# Autodesk Inventor assembly: BATTERY ASSEMBLY
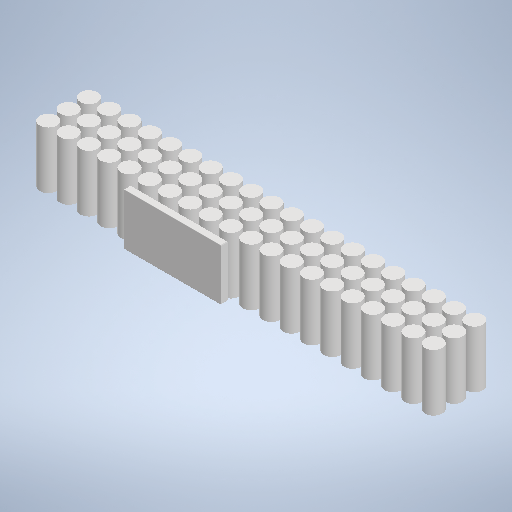
[picture p0: Inventor's stored thumbnail of the model, 512x512]
Saved by Autodesk Inventor 2025.2 (Build 292293000, 293)
## iProperties
Created: 2025-03-22
Part Number: BATTERY ASSEMBLY
Document SubType Name: Assembly
Designer: Mathias
Author: Mathias
## Documents named in this file (3)
- C:\Users\Mathias\Desktop\Projekt Olkassa\Autodesk-inventor-filesharing\BATTERY ASSEMBLY.iam
- C:\Users\Mathias\Desktop\Projekt Olkassa\Autodesk-inventor-filesharing\21700.ipt
- C:\Users\Mathias\Desktop\Projekt Olkassa\Autodesk-inventor-filesharing\BMS.ipt
## Components (61 placed, 2 different names)
1. BMS:1
2. 21700:1
3. 21700:2
4. 21700:3
5. 21700:4
6. 21700:5
7. 21700:6
8. 21700:7
9. 21700:8
10. 21700:9
11. 21700:10
12. 21700:11
13. 21700:12
14. 21700:13
15. 21700:14
16. 21700:15
17. 21700:16
18. 21700:17
19. 21700:18
20. 21700:19
21. 21700:20
22. 21700:21
23. 21700:22
24. 21700:23
25. 21700:24
26. 21700:25
27. 21700:26
28. 21700:27
29. 21700:28
30. 21700:29
31. 21700:30
32. 21700:31
33. 21700:32
34. 21700:33
35. 21700:34
36. 21700:35
37. 21700:36
38. 21700:37
39. 21700:38
40. 21700:39
41. 21700:40
42. 21700:41
43. 21700:42
44. 21700:43
45. 21700:44
46. 21700:45
47. 21700:46
48. 21700:47
49. 21700:48
50. 21700:49
51. 21700:50
52. 21700:51
53. 21700:52
54. 21700:53
55. 21700:54
56. 21700:55
57. 21700:56
58. 21700:57
59. 21700:58
60. 21700:59
61. 21700:60
## Component patterns: (60 elements, first: 21700:1)
